# Autodesk Inventor assembly: Ares
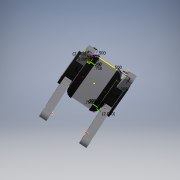
[picture p0: Inventor's stored thumbnail of the model, 180x180]
Saved by Autodesk Inventor 2018.2 (Build 222227000, 227)
## iProperties
Created: 2018-02-01
Part Number: Ares
Document SubType Name: Assembly
Designer: MIABo
Author: MIABo
## Documents named in this file (4)
- C:\Users\MIABo\OneDrive\Documents\GitHub\Ares\Ares.iam
- C:\Users\MIABo\OneDrive\Documents\GitHub\Ares\SUspension mounting.ipt
- C:\Users\MIABo\OneDrive\Documents\GitHub\Ares\Frame.ipt
- C:\Users\MIABo\OneDrive\Documents\GitHub\Ares\Leg Assembly.ipt
## Components (7 placed, 3 different names)
1. SUspension mounting:1 — Mate:1, Mate:2, Mate:3, Mate:7, Rotational:1, Rotational:2
2. Frame:1 — Mate:1, Mate:2, Mate:3, Mate:4, Mate:5, Mate:6, Mate:7
3. SUspension mounting:2 — Mate:4, Mate:5, Mate:6, Rotational:3, Rotational:4
4. Leg Assembly:1 — Rotational:4
5. Leg Assembly:2 — Rotational:2
6. Leg Assembly:3 — Rotational:1
7. Leg Assembly:4 — Rotational:3
## Relationships (11: Mate 7, RevoluteJoint 4)
- Mate:1: SUspension mounting:1 ↔ Frame:1
- Mate:2: SUspension mounting:1 ↔ Frame:1
- Mate:3: SUspension mounting:1 ↔ Frame:1
- Mate:4: Frame:1 ↔ SUspension mounting:2
- Mate:5: Frame:1 ↔ SUspension mounting:2
- Mate:6: Frame:1 ↔ SUspension mounting:2
- Mate:7: SUspension mounting:1 ↔ Frame:1
- Rotational:1 [RevoluteJoint]: SUspension mounting:1 ↔ Leg Assembly:3
- Rotational:2 [RevoluteJoint]: SUspension mounting:1 ↔ Leg Assembly:2
- Rotational:3 [RevoluteJoint] (1.27 mm): SUspension mounting:2 ↔ Leg Assembly:4
- Rotational:4 [RevoluteJoint] (1.27 mm): SUspension mounting:2 ↔ Leg Assembly:1
